# Autodesk Inventor assembly: shooter
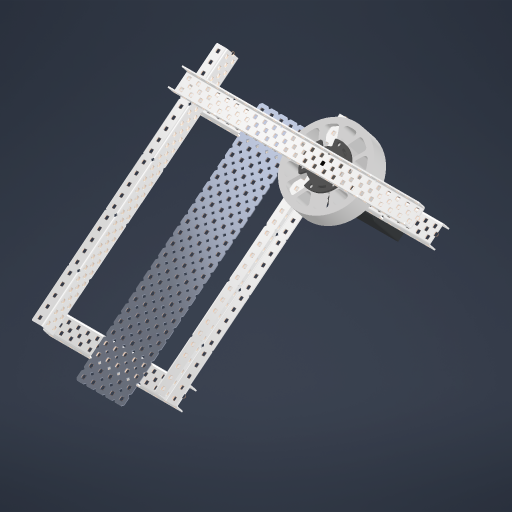
[picture p0: Inventor's stored thumbnail of the model, 512x512]
Saved by Autodesk Inventor 2023 (Build 270158000, 158)
## iProperties
Created: 2023-03-01
Part Number: shooter
Document SubType Name: Assembly
Designer: Windows Macbook
Author: Windows Macbook
## Documents named in this file (10)
- C:\Users\Windows Macbook\Desktop\VRC-SPIN-UP\Inventor\Assembly\Pre Worlds\shooter.iam
- C:\Users\Windows Macbook\Desktop\VRC-SPIN-UP\Inventor\Structure\C Channel\Aluminum 1x2x1\Alu C 1x2x1x14.ipt
- C:\Users\Windows Macbook\Desktop\VRC-SPIN-UP\Inventor\Structure\Plate\Steel\Steel Plate 5x25.ipt
- C:\Users\Windows Macbook\Desktop\VRC-SPIN-UP\Inventor\Motion\Shaft LS\Bearing Flat.ipt
- C:\Users\Windows Macbook\Desktop\VRC-SPIN-UP\Inventor\Motion\Spacers\Spacer Nylon .313 OD.ipt
- C:\Users\Windows Macbook\Desktop\VRC-SPIN-UP\Inventor\Motion\Shaft LS\Shaft Collar Rubber.ipt
- C:\Users\Windows Macbook\Desktop\VRC-SPIN-UP\Inventor\Motion\Wheels\Flex Wheels\4 Flex, LS.iam
- C:\Users\Windows Macbook\Desktop\VRC-SPIN-UP\Inventor\Structure\C Channel\Aluminum 1x2x1\Alu C 1x2x1x25.ipt
- C:\Users\Windows Macbook\Desktop\VRC-SPIN-UP\Inventor\Electronics\V5 Simple Motor.ipt
- C:\Users\Windows Macbook\Desktop\VRC-SPIN-UP\Inventor\Motion\Spacers\Spacer Nylon .313 OD\NSpacer .313 OD x .500.ipt
## Components (12 placed, 8 different names)
1. Alu C 1x2x1x14:1 — Insert:7, Insert:8, Insert:59, Insert:60, Insert:61, Insert:62
2. Alu C 1x2x1x25:1 — Insert:48, Insert:49, Insert:50, Insert:63, Insert:64
3. Steel Plate 5x25:1 — Insert:7, Insert:8
4. 4 Flex, LS:1 [sub-assembly] — Insert:48
5. Bearing Flat:6 — Insert:49, Insert:50, Insert:51, Insert:52, Insert:53
6. Shaft Collar Rubber:11 — Insert:51
7. V5 Simple Motor:1 — Insert:52, Insert:53
8. Alu C 1x2x1x25:2 — Insert:57, Insert:58
9. NSpacer .313 OD x .500:3 — Insert:57, Insert:66
10. NSpacer .313 OD x .500:4 — Insert:58, Insert:65
11. Alu C 1x2x1x25:3 — Insert:61, Insert:62
12. Alu C 1x2x1x25:4 — Insert:59, Insert:60, Insert:63, Insert:64, Insert:65, Insert:66
## Relationships (18: Insert 18)
- Insert:7: Alu C 1x2x1x14:1 ↔ Steel Plate 5x25:1
- Insert:8: Alu C 1x2x1x14:1 ↔ Steel Plate 5x25:1
- Insert:48: Alu C 1x2x1x25:1 ↔ 4 Flex, LS:1
- Insert:49: Alu C 1x2x1x25:1 ↔ Bearing Flat:6
- Insert:50: Alu C 1x2x1x25:1 ↔ Bearing Flat:6
- Insert:51 (0.889 mm): Bearing Flat:6 ↔ Shaft Collar Rubber:11
- Insert:52: Bearing Flat:6 ↔ V5 Simple Motor:1
- Insert:53: Bearing Flat:6 ↔ V5 Simple Motor:1
- Insert:57: Alu C 1x2x1x25:2 ↔ NSpacer .313 OD x .500:3
- Insert:58: Alu C 1x2x1x25:2 ↔ NSpacer .313 OD x .500:4
- Insert:59: Alu C 1x2x1x14:1 ↔ Alu C 1x2x1x25:4
- Insert:60: Alu C 1x2x1x14:1 ↔ Alu C 1x2x1x25:4
- Insert:61: Alu C 1x2x1x14:1 ↔ Alu C 1x2x1x25:3
- Insert:62: Alu C 1x2x1x14:1 ↔ Alu C 1x2x1x25:3
- Insert:63: Alu C 1x2x1x25:1 ↔ Alu C 1x2x1x25:4
- Insert:64: Alu C 1x2x1x25:1 ↔ Alu C 1x2x1x25:4
- Insert:65: NSpacer .313 OD x .500:4 ↔ Alu C 1x2x1x25:4
- Insert:66: NSpacer .313 OD x .500:3 ↔ Alu C 1x2x1x25:4
